# Autodesk Inventor assembly: Mechanics Assembly
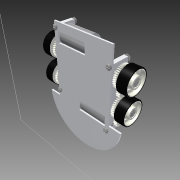
[picture p0: Inventor's stored thumbnail of the model, 180x180]
Saved by Autodesk Inventor 2014 (Build 180170000, 170)
## iProperties
Created: 2013-09-11
Part Number: Mechanics Assembly
Document SubType Name: Assembly
Designer: Brandon
Author: Brandon
## Documents named in this file (18)
- C:\Users\Brandon\Dropbox\engineering\IEEEUCR-MM-2014\hardware\Reference_Mouse_v1\3D\Mechanics Assembly.iam
- C:\Users\Brandon\Dropbox\engineering\IEEEUCR-MM-2014\hardware\Reference_Mouse_v1\3D\Wheel.ipt
- C:\Users\Brandon\Dropbox\engineering\IEEEUCR-MM-2014\hardware\Reference_Mouse_v1\3D\Wheel2Wheel.ipt
- C:\Users\Brandon\Dropbox\engineering\IEEEUCR-MM-2014\hardware\Reference_Mouse_v1\3D\Wheel_MIR.ipt
- C:\Users\Brandon\Dropbox\engineering\IEEEUCR-MM-2014\hardware\Reference_Mouse_v1\3D\mount.ipt
- C:\Users\Brandon\Dropbox\engineering\IEEEUCR-MM-2014\hardware\Reference_Mouse_v1\3D\gear motor.ipt
- C:\Users\Brandon\Dropbox\engineering\IEEEUCR-MM-2014\hardware\Reference_Mouse_v1\3D\idler shaft.ipt
- C:\Users\Brandon\Dropbox\engineering\IEEEUCR-MM-2014\hardware\Reference_Mouse_v1\3D\PCB.ipt
- C:\Users\Brandon\Dropbox\engineering\IEEEUCR-MM-2014\hardware\Reference_Mouse_v1\3D\motor.ipt
- C:\Users\Brandon\Dropbox\engineering\IEEEUCR-MM-2014\hardware\Reference_Mouse_v1\3D\IMPORTED COMPONENTS\7804K129\7804K129.IPT
- C:\Users\Brandon\Dropbox\engineering\IEEEUCR-MM-2014\hardware\Reference_Mouse_v1\3D\IMPORTED COMPONENTS\90710A025\90710A025.IPT
- C:\Users\Brandon\Dropbox\engineering\IEEEUCR-MM-2014\hardware\Reference_Mouse_v1\3D\IMPORTED COMPONENTS\92095A197\92095A197.IPT
- C:\Users\Brandon\Dropbox\engineering\IEEEUCR-MM-2014\hardware\Reference_Mouse_v1\3D\IMPORTED COMPONENTS\90576A103\90576A103.IPT
- C:\Users\Brandon\Dropbox\engineering\IEEEUCR-MM-2014\hardware\Reference_Mouse_v1\3D\Tire.ipt
- C:\Users\Brandon\Dropbox\engineering\IEEEUCR-MM-2014\hardware\Reference_Mouse_v1\3D\MCMASTERCARR PARTS\IMPORTED COMPONENTS\92010A003\92010A003.IPT
- C:\Users\Brandon\Dropbox\engineering\IEEEUCR-MM-2014\hardware\Reference_Mouse_v1\3D\McMasterCarr Parts\IMPORTED COMPONENTS\92005A077\92005A077.IPT
- C:\Users\Brandon\Dropbox\engineering\IEEEUCR-MM-2014\hardware\Reference_Mouse_v1\3D\MCMASTERCARR PARTS\IMPORTED COMPONENTS\96817A113\96817A113.IPT
- C:\Users\Brandon\Dropbox\engineering\IEEEUCR-MM-2014\hardware\Reference_Mouse_v1\3D\MCMASTERCARR PARTS\IMPORTED COMPONENTS\91166A170\91166A170.IPT
## Components (58 placed, 26 different names)
1. LF Wheel — Rotation:3, Rotational:2, Rotation:5, Insert:19, Insert:23, Mate:28
2. Left Idler — Mate:1, Rotation:3, Rotational:3, Rotation:4
3. LB Wheel — Rotational:1, Rotation:4, Insert:20, Insert:24, Mate:29
4. Left Mount — Rotational:1, Rotational:2, Rotational:3, Rotational:4, Flush:2, Mate:5, Mate:8, Mate:9, Angle:1, Insert:1, Mate:22, Mate:23, Mate:24, Insert:3, Insert:4, Insert:13, Insert:14, Insert:29, Insert:30, Insert:31, Insert:32, Insert:33, Insert:34
5. Left Motor Output — Rotational:4, Rotation:5
6. RB Wheel — Insert:21, Insert:26, Mate:27
7. Right Idler
8. RF Wheel — Insert:22, Insert:25
9. Right Mount — Mate:3, Mate:6, Mate:7, Mate:10, Mate:18, Insert:2, Mate:21, Mate:25, Mate:26, Insert:5, Insert:6, Insert:11, Insert:12, Insert:27, Insert:28, Insert:39, Insert:40, Insert:41, Insert:42
10. Right Motor Output
11. Idler Shaft — Mate:14, Mate:15, Mate:16, Mate:17
12. PCB — Flush:3, Mate:19, Mate:20, Mate:23, Mate:24, Mate:25, Mate:26, Insert:7, Insert:8, Insert:9, Insert:10
13. L motor — Insert:1, Mate:22
14. R motor — Insert:2, Mate:21
15. LF Bearing — Insert:3, Insert:17
16. RF Bearing — Insert:5, Insert:16
17. RB Bearing — Insert:6, Insert:15
18. LB Bearing — Insert:4, Insert:18
19. 92005A077:5 — Insert:8
20. 92005A077:6 — Insert:7
21. 92005A077:7 — Insert:9
22. 92005A077:8 — Insert:10
23. 90710A025:1 — Insert:11
24. 90710A025:2 — Insert:12
25. 90710A025:3 — Insert:14
26. 90710A025:4 — Insert:13
27. 92095A197:1 — Insert:15
28. 92095A197:2 — Insert:17
29. 92095A197:3 — Insert:18
30. 92095A197:4 — Insert:16
31. 90576A103:1 — Insert:20, Mate:29
32. 90576A103:2 — Insert:19, Mate:28
33. 90576A103:3 — Insert:22
34. 90576A103:4 — Insert:21, Mate:27
35. Tire:1 — Flush:4, Insert:23
36. Tire:2 — Insert:24
37. Tire:3 — Insert:26
38. Tire:4 — Insert:25
39. 92010A003:1 — Insert:28
40. 92010A003:2 — Insert:27
41. 92010A003:3 — Insert:29
42. 92010A003:4 — Insert:30
43. 96817A113:1 — Insert:38
44. 96817A113:2 — Insert:37
45. 96817A113:3 — Insert:36
46. 96817A113:4 — Insert:35
47. 96817A113:5 — Insert:46
48. 96817A113:6 — Insert:45
49. 96817A113:7 — Insert:44
50. 96817A113:8 — Insert:43
51. 91166A170:1 — Insert:34, Insert:38
52. 91166A170:2 — Insert:33, Insert:37
53. 91166A170:3 — Insert:32, Insert:35
54. 91166A170:4 — Insert:31, Insert:36
55. 91166A170:5 — Insert:39, Insert:43
56. 91166A170:6 — Insert:40, Insert:45
57. 91166A170:7 — Insert:41, Insert:46
58. 91166A170:8 — Insert:42, Insert:44
## Relationships (91: Insert 46, Mate 27, RevoluteJoint 8, RelateRotation 6, Flush 3, Angle 1)
- Mate:1: Left Idler
- Rotation:3 [RelateRotation] (0.667 ul): LF Wheel ↔ Left Idler
- Rotational:1 [RevoluteJoint]: LB Wheel ↔ Left Mount
- Rotational:2 [RevoluteJoint]: LF Wheel ↔ Left Mount
- Rotational:3 [RevoluteJoint] (-1.25 mm): Left Idler ↔ Left Mount
- Rotation:4 [RelateRotation] (0.6667 ul): Left Idler ↔ LB Wheel
- Rotational:4 [RevoluteJoint] (0.2 mm): Left Mount ↔ Left Motor Output
- Rotation:5 [RelateRotation] (2 ul): LF Wheel ↔ Left Motor Output
- Flush:2 (-24.5 mm): Left Mount
- [RelateRotation] (0.667 ul): RB Wheel ↔ Right Idler
- [RevoluteJoint]: RF Wheel ↔ Right Mount
- [RevoluteJoint]: RB Wheel ↔ Right Mount
- [RevoluteJoint] (-1.25 mm): Right Idler ↔ Right Mount
- [RelateRotation] (0.6667 ul): Right Idler ↔ RF Wheel
- [RevoluteJoint] (0.2 mm): Right Mount ↔ Right Motor Output
- [RelateRotation] (2 ul): RB Wheel ↔ Right Motor Output
- Mate:3 (24.5 mm): Right Mount
- Mate:5: Left Mount
- Mate:6: Right Mount
- Mate:7 (4 mm): Right Mount
- Mate:8 (4 mm): Left Mount
- Mate:9: Left Mount
- Mate:10: Right Mount
- Mate:11
- Mate:12
- Mate:13
- Mate:14: Idler Shaft
- Mate:15: Idler Shaft
- Mate:16: Idler Shaft
- Mate:17: Idler Shaft
- Mate:18: Right Mount
- Angle:1 (0 deg): Left Mount
- Flush:3: PCB
- Mate:19 (-14 mm): PCB
- Mate:20: PCB
- Insert:1: Left Mount ↔ L motor
- Insert:2: Right Mount ↔ R motor
- Mate:21: Right Mount ↔ R motor
- Mate:22: Left Mount ↔ L motor
- Mate:23: Left Mount ↔ PCB
- Mate:24: Left Mount ↔ PCB
- Mate:25: Right Mount ↔ PCB
- Mate:26: Right Mount ↔ PCB
- Insert:3 (0.1 mm): Left Mount ↔ LF Bearing
- Insert:4 (0.1 mm): Left Mount ↔ LB Bearing
- Insert:5 (0.1 mm): Right Mount ↔ RF Bearing
- Insert:6 (0.1 mm): Right Mount ↔ RB Bearing
- Insert:7: PCB ↔ 92005A077:6
- Insert:8: PCB ↔ 92005A077:5
- Insert:9: PCB ↔ 92005A077:7
- Insert:10: PCB ↔ 92005A077:8
- Insert:11: Right Mount ↔ 90710A025:1
- Insert:12: Right Mount ↔ 90710A025:2
- Insert:13: Left Mount ↔ 90710A025:4
- Insert:14: Left Mount ↔ 90710A025:3
- Insert:15: RB Bearing ↔ 92095A197:1
- Insert:16: RF Bearing ↔ 92095A197:4
- Insert:17: LF Bearing ↔ 92095A197:2
- Insert:18: LB Bearing ↔ 92095A197:3
- Insert:19: LF Wheel ↔ 90576A103:2
- Insert:20: LB Wheel ↔ 90576A103:1
- Insert:21: RB Wheel ↔ 90576A103:4
- Insert:22: RF Wheel ↔ 90576A103:3
- Flush:4: Tire:1
- Insert:23: LF Wheel ↔ Tire:1
- Insert:24: LB Wheel ↔ Tire:2
- Insert:25: RF Wheel ↔ Tire:4
- Insert:26: RB Wheel ↔ Tire:3
- Mate:27: RB Wheel ↔ 90576A103:4
- Mate:28: LF Wheel ↔ 90576A103:2
- Mate:29: LB Wheel ↔ 90576A103:1
- Insert:27 (0.1 mm): Right Mount ↔ 92010A003:2
- Insert:28 (0.1 mm): Right Mount ↔ 92010A003:1
- Insert:29 (0.1 mm): Left Mount ↔ 92010A003:3
- Insert:30 (0.1 mm): Left Mount ↔ 92010A003:4
- Insert:31: Left Mount ↔ 91166A170:4
- Insert:32: Left Mount ↔ 91166A170:3
- Insert:33: Left Mount ↔ 91166A170:2
- Insert:34: Left Mount ↔ 91166A170:1
- Insert:35: 96817A113:4 ↔ 91166A170:3
- Insert:36: 96817A113:3 ↔ 91166A170:4
- Insert:37: 96817A113:2 ↔ 91166A170:2
- Insert:38: 96817A113:1 ↔ 91166A170:1
- Insert:39: Right Mount ↔ 91166A170:5
- Insert:40: Right Mount ↔ 91166A170:6
- Insert:41: Right Mount ↔ 91166A170:7
- Insert:42: Right Mount ↔ 91166A170:8
- Insert:43: 96817A113:8 ↔ 91166A170:5
- Insert:44: 96817A113:7 ↔ 91166A170:8
- Insert:45: 96817A113:6 ↔ 91166A170:6
- Insert:46: 96817A113:5 ↔ 91166A170:7
## Named parameters: d62_d57 = 0.2 mm, d63_d58 = -4.554369 deg, d64_d59 = 2, d65_d35 = 0 mm, d66_d36 = 61.162763 deg, d67_d39 = 0 mm, d68_d40 = -28.868955 deg, d69_d47 = -1.25 mm, d70_d48 = 9.663939 deg, d71_d55 = 0.666667, d72_d9 = 0.667
